# Autodesk Inventor assembly: RIGHT RAIL ASSY
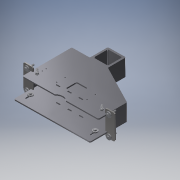
[picture p0: Inventor's stored thumbnail of the model, 180x180]
Saved by Autodesk Inventor 2018 (Build 220112000, 112)
## iProperties
Created: 2018-10-15
Part Number: RIGHT RAIL ASSY
Material: Genérico
Document SubType Name: Assembly
Designer: Toshiba
Author: Toshiba
## Documents named in this file (7)
- C:\U\Semestre Primavera 2018\Diseño de sistemas mecánicos\CNC\DiseñoCNC\Gantry\RIGHT RAIL ASSY.iam
- C:\U\Semestre Primavera 2018\Diseño de sistemas mecánicos\CNC\DiseñoCNC\Gantry\INTERNAL SIDE PLATE.ipt
- C:\U\Semestre Primavera 2018\Diseño de sistemas mecánicos\CNC\DiseñoCNC\Gantry\INTERNAL FRAME.ipt
- C:\U\Semestre Primavera 2018\Diseño de sistemas mecánicos\CNC\DiseñoCNC\Gantry\EXTERNAL SIDE PLATE.ipt
- C:\U\Semestre Primavera 2018\Diseño de sistemas mecánicos\CNC\DiseñoCNC\Gantry\SIDE BEARING GUIDE.ipt
- C:\U\Semestre Primavera 2018\Diseño de sistemas mecánicos\CNC\DiseñoCNC\Gantry\BEARING SYSTEM.iam
- C:\U\Semestre Primavera 2018\Diseño de sistemas mecánicos\CNC\DiseñoCNC\Gantry\FLANGE NUT M8.ipt
## Components (21 placed, 6 different names)
1. INTERNAL SIDE PLATE:1 — Coincidencia:1, Coincidencia:2, Coincidencia:3, Insertar:5, Insertar:6, Insertar:9, Insertar:10
2. INTERNAL FRAME:1 — Coincidencia:1, Coincidencia:2, Coincidencia:3, Coincidencia:4, Coincidencia:5, Coincidencia:6
3. EXTERNAL SIDE PLATE:1 — Coincidencia:4, Coincidencia:5, Coincidencia:6, Coincidencia:7, Nivelación:1, Coincidencia:8, Coincidencia:9, Coincidencia:11, Insertar:1, Insertar:2, Insertar:13, Insertar:14
4. SIDE BEARING GUIDE:1 — Coincidencia:7, Nivelación:1, Coincidencia:8, Coincidencia:10, Insertar:7, Insertar:8, Insertar:11, Insertar:12
5. SIDE BEARING GUIDE:2 — Coincidencia:9, Coincidencia:10, Coincidencia:11, Insertar:3, Insertar:4, Insertar:15, Insertar:16
6. BEARING SYSTEM:1 [sub-assembly] — Insertar:7
7. BEARING SYSTEM:2 [sub-assembly] — Insertar:8
8. BEARING SYSTEM:3 [sub-assembly] — Insertar:4
9. BEARING SYSTEM:4 [sub-assembly] — Insertar:3
10. BEARING SYSTEM:5 [sub-assembly] — Insertar:6
11. BEARING SYSTEM:6 [sub-assembly] — Insertar:5
12. BEARING SYSTEM:7 [sub-assembly] — Insertar:1
13. BEARING SYSTEM:8 [sub-assembly] — Insertar:2
14. FLANGE NUT M8:1 — Insertar:13
15. FLANGE NUT M8:2 — Insertar:14
16. FLANGE NUT M8:3 — Insertar:12
17. FLANGE NUT M8:4 — Insertar:11
18. FLANGE NUT M8:5 — Insertar:15
19. FLANGE NUT M8:6 — Insertar:16
20. FLANGE NUT M8:7 — Insertar:9
21. FLANGE NUT M8:8 — Insertar:10
## Relationships (28: Insert 16, Mate 11, Flush 1)
- Coincidencia:1 [Mate]: INTERNAL SIDE PLATE:1 ↔ INTERNAL FRAME:1
- Coincidencia:2 [Mate]: INTERNAL SIDE PLATE:1 ↔ INTERNAL FRAME:1
- Coincidencia:3 [Mate]: INTERNAL SIDE PLATE:1 ↔ INTERNAL FRAME:1
- Coincidencia:4 [Mate]: INTERNAL FRAME:1 ↔ EXTERNAL SIDE PLATE:1
- Coincidencia:5 [Mate]: INTERNAL FRAME:1 ↔ EXTERNAL SIDE PLATE:1
- Coincidencia:6 [Mate]: INTERNAL FRAME:1 ↔ EXTERNAL SIDE PLATE:1
- Coincidencia:7 [Mate]: EXTERNAL SIDE PLATE:1 ↔ SIDE BEARING GUIDE:1
- Nivelación:1 [Flush] (-21.5 mm): EXTERNAL SIDE PLATE:1 ↔ SIDE BEARING GUIDE:1
- Coincidencia:8 [Mate]: EXTERNAL SIDE PLATE:1 ↔ SIDE BEARING GUIDE:1
- Coincidencia:9 [Mate]: EXTERNAL SIDE PLATE:1 ↔ SIDE BEARING GUIDE:2
- Coincidencia:10 [Mate]: SIDE BEARING GUIDE:1 ↔ SIDE BEARING GUIDE:2
- Coincidencia:11 [Mate]: EXTERNAL SIDE PLATE:1 ↔ SIDE BEARING GUIDE:2
- Insertar:1: EXTERNAL SIDE PLATE:1 ↔ BEARING SYSTEM:7
- Insertar:2: EXTERNAL SIDE PLATE:1 ↔ BEARING SYSTEM:8
- Insertar:3: SIDE BEARING GUIDE:2 ↔ BEARING SYSTEM:4
- Insertar:4: SIDE BEARING GUIDE:2 ↔ BEARING SYSTEM:3
- Insertar:5: INTERNAL SIDE PLATE:1 ↔ BEARING SYSTEM:6
- Insertar:6: INTERNAL SIDE PLATE:1 ↔ BEARING SYSTEM:5
- Insertar:7: SIDE BEARING GUIDE:1 ↔ BEARING SYSTEM:1
- Insertar:8: SIDE BEARING GUIDE:1 ↔ BEARING SYSTEM:2
- Insertar:9: INTERNAL SIDE PLATE:1 ↔ FLANGE NUT M8:7
- Insertar:10: INTERNAL SIDE PLATE:1 ↔ FLANGE NUT M8:8
- Insertar:11: SIDE BEARING GUIDE:1 ↔ FLANGE NUT M8:4
- Insertar:12: SIDE BEARING GUIDE:1 ↔ FLANGE NUT M8:3
- Insertar:13: EXTERNAL SIDE PLATE:1 ↔ FLANGE NUT M8:1
- Insertar:14: EXTERNAL SIDE PLATE:1 ↔ FLANGE NUT M8:2
- Insertar:15: SIDE BEARING GUIDE:2 ↔ FLANGE NUT M8:5
- Insertar:16: SIDE BEARING GUIDE:2 ↔ FLANGE NUT M8:6
